# Autodesk Inventor assembly: linear bearing shroud
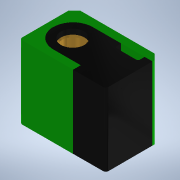
[picture p0: Inventor's stored thumbnail of the model, 180x180]
Saved by Autodesk Inventor 2020 (Build 240168000, 168)
## iProperties
Created: 2021-02-25
Part Number: linear bearing shroud
Document SubType Name: Assembly
Designer: AOB
Mass: 42.3762 g
Surface Area: 103.335 cm^2
Volume: 13.0352 cm^3
Density: 3.25091 g/cm^3
Author: AOB
## Documents named in this file (4)
- C:\Users\marti\Documents\Inventor\ProjectBoron\linear bearing shroud.iam
- C:\Users\marti\Documents\Inventor\ProjectBoron\linear bearing shroud-right half.ipt
- C:\Users\marti\Documents\Inventor\ProjectBoron\shroud left half.ipt
- C:\Users\marti\Documents\Inventor\ProjectBoron\lm8uu-graphite.ipt
## Components (3 placed, 3 different names)
1. linear bearing shroud-right half:1 — Flush:1, Rigid:1
2. shroud left half:1 — Flush:1, Rigid:1, Mate:1, Mate:2
3. lm8uu-graphite:1 — Mate:1, Mate:2
## Relationships (4: Mate 2, Flush 1, WeldJoint 1)
- Flush:1: linear bearing shroud-right half:1 ↔ shroud left half:1
- Rigid:1 [WeldJoint]: linear bearing shroud-right half:1 ↔ shroud left half:1
- Mate:1: shroud left half:1 ↔ lm8uu-graphite:1
- Mate:2: shroud left half:1 ↔ lm8uu-graphite:1
